# Autodesk Inventor assembly: Сборка1
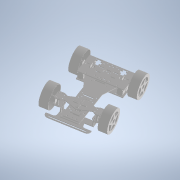
[picture p0: Inventor's stored thumbnail of the model, 180x180]
Saved by Autodesk Inventor 2022 (Build 260153000, 153)
## iProperties
Created: 2022-07-10
Part Number: Сборка1
Document SubType Name: Assembly
Designer: Константин
Author: Константин
## Documents named in this file (16)
- C:\Users\Константин\Desktop\практика галактика\Сборка1.iam
- C:\Users\Константин\Downloads\мотор.ipt
- C:\Users\Константин\Downloads\Рама.ipt
- C:\Users\Константин\Downloads\Ось.ipt
- C:\Users\Константин\Downloads\Крепеж.ipt
- C:\Users\Константин\Downloads\Звезда.ipt
- C:\Users\Константин\Downloads\Задняя часть.ipt
- C:\Users\Константин\Downloads\Бампер.ipt
- C:\Users\Константин\Downloads\m3x29.ipt
- C:\Users\Константин\Desktop\практика галактика\Колесо красивое.ipt
- C:\Users\Константин\Desktop\практика галактика\Крепеж колеса.ipt
- C:\Users\Константин\Desktop\практика галактика\Крепежная деталь.ipt
- C:\Users\Константин\Desktop\практика галактика\Кусок металла.ipt
- C:\Users\Константин\Desktop\практика галактика\Пластинка шасси.ipt
- C:\Users\Константин\Desktop\практика галактика\Сервопривод.ipt
- C:\Users\Константин\Desktop\практика галактика\Колесо красивое(для мотора).ipt
## Components (32 placed, 15 different names)
1. мотор:1 — Совмещение:61, Совмещение:62, Совмещение:63, Совмещение:64, Совмещение:65, Совмещение:72, Совмещение:79, Совмещение:80, Совмещение:81
2. Рама:1 — Совмещение:28, Совмещение:29, Совмещение:30, Угол:1, С поворотом:4, С поворотом:5, Совмещение:73, Совмещение:74, Совмещение:75
3. Ось:1 — Совмещение:1, Совмещение:27, Угол:1, Совмещение:50, С поворотом:1, Совмещение:51, Совмещение:55, Совмещение:56, Совмещение:57, Совмещение:58, Совмещение:59
4. Крепеж:1 — Совмещение:67, Совмещение:69, Совмещение:76, Совмещение:77
5. Звезда:1 — Совмещение:1, Совмещение:27, Совмещение:31, Совмещение:32
6. Задняя часть:1 — Совмещение:65, Совмещение:70, С поворотом:3, Совмещение:73, Совмещение:74, Совмещение:75, Угол:2
7. Бампер:1 — С поворотом:4, С поворотом:5
8. Крепеж колеса:1 — Совмещение:57, Совмещение:58, Совмещение:60, Совмещение:85
9. Сервопривод:1 — Совмещение:28, Совмещение:29, Совмещение:30, Совмещение:31, Совмещение:32
10. Крепежная деталь:2 — Совмещение:8, Совмещение:9, Совмещение:10, Совмещение:11, Совмещение:60
11. Кусок металла:4 — Совмещение:36, Совмещение:41, Совмещение:44, Совмещение:47
12. Кусок металла:5 — Совмещение:37, Совмещение:38, Совмещение:45, Совмещение:46
13. Кусок металла:7 — Совмещение:8, Совмещение:10
14. Кусок металла:9 — Совмещение:9, Совмещение:11
15. Крепежная деталь:3
16. Кусок металла:10 — Совмещение:35, Совмещение:39, Совмещение:43, Совмещение:49
17. Кусок металла:11 — Совмещение:34, Совмещение:40, Совмещение:42, Совмещение:48
18. Кусок металла:12 — Совмещение:50, С поворотом:1
19. Кусок металла:13 — Совмещение:51
20. Пластинка шасси:3 — Совмещение:34, Совмещение:35, Совмещение:36, Совмещение:37, Совмещение:38, Совмещение:39, Совмещение:40, Совмещение:41, Совмещение:42, Совмещение:43, Совмещение:44, Совмещение:45, Совмещение:46, Совмещение:47, Совмещение:48, Совмещение:49
21. Крепеж колеса:2 — Совмещение:55, Совмещение:56, Совмещение:59, Совмещение:87
22. Крепеж:2 — Совмещение:61, Совмещение:63
23. мотор:2 — Совмещение:66, Совмещение:67, Совмещение:68, Совмещение:69, Совмещение:70, Совмещение:82, Совмещение:83, Совмещение:84
24. Крепеж:3 — Совмещение:62, Совмещение:64, Совмещение:78
25. Крепеж:4 — Совмещение:66, Совмещение:68
26. m3x29:4 — Совмещение:72, Совмещение:78
27. Задняя часть:2 — С поворотом:3, Угол:2
28. m3x29:5 — Совмещение:76, Совмещение:77
29. Колесо красивое(для мотора):1 — Совмещение:79, Совмещение:80, Совмещение:81
30. Колесо красивое:1 — Совмещение:85
31. Колесо красивое(для мотора):2 — Совмещение:82, Совмещение:83, Совмещение:84, Заподлицо:1
32. Колесо красивое:2 — Совмещение:87, Заподлицо:1
## Relationships (79: Mate 68, CylindricalJoint 4, RevoluteJoint 4, Angle 2, Flush 1)
- Совмещение:1 [Mate]: Ось:1 ↔ Звезда:1
- [CylindricalJoint]: Крепежная деталь:2 ↔ Кусок металла:4
- [CylindricalJoint]: Крепежная деталь:2 ↔ Кусок металла:5
- [Mate]: Крепежная деталь:2 ↔ Кусок металла:5
- [Mate]: Крепежная деталь:2 ↔ Кусок металла:4
- Совмещение:8 [Mate]: Крепежная деталь:2 ↔ Кусок металла:7
- Совмещение:9 [Mate]: Крепежная деталь:2 ↔ Кусок металла:9
- Совмещение:10 [Mate]: Крепежная деталь:2 ↔ Кусок металла:7
- Совмещение:11 [Mate]: Крепежная деталь:2 ↔ Кусок металла:9
- [CylindricalJoint]: Крепежная деталь:3 ↔ Кусок металла:10
- [CylindricalJoint]: Крепежная деталь:3 ↔ Кусок металла:11
- [Mate]: Крепежная деталь:3 ↔ Кусок металла:11
- [Mate]: Крепежная деталь:3 ↔ Кусок металла:10
- [Mate]: Крепежная деталь:3 ↔ Кусок металла:12
- [Mate]: Крепежная деталь:3 ↔ Кусок металла:13
- [Mate]: Крепежная деталь:3 ↔ Кусок металла:12
- [Mate]: Крепежная деталь:3 ↔ Кусок металла:13
- Совмещение:27 [Mate]: Ось:1 ↔ Звезда:1
- Совмещение:28 [Mate]: Рама:1 ↔ Сервопривод:1
- Совмещение:29 [Mate]: Рама:1 ↔ Сервопривод:1
- Совмещение:30 [Mate]: Рама:1 ↔ Сервопривод:1
- Совмещение:31 [Mate]: Звезда:1 ↔ Сервопривод:1
- Совмещение:32 [Mate]: Звезда:1 ↔ Сервопривод:1
- Угол:1 [Angle] (0 deg): Рама:1 ↔ Ось:1
- Совмещение:34 [Mate]: Кусок металла:11 ↔ Пластинка шасси:3
- Совмещение:35 [Mate]: Кусок металла:10 ↔ Пластинка шасси:3
- Совмещение:36 [Mate]: Кусок металла:4 ↔ Пластинка шасси:3
- Совмещение:37 [Mate]: Кусок металла:5 ↔ Пластинка шасси:3
- Совмещение:38 [Mate]: Кусок металла:5 ↔ Пластинка шасси:3
- Совмещение:39 [Mate]: Кусок металла:10 ↔ Пластинка шасси:3
- Совмещение:40 [Mate]: Кусок металла:11 ↔ Пластинка шасси:3
- Совмещение:41 [Mate]: Кусок металла:4 ↔ Пластинка шасси:3
- Совмещение:42 [Mate]: Кусок металла:11 ↔ Пластинка шасси:3
- Совмещение:43 [Mate]: Кусок металла:10 ↔ Пластинка шасси:3
- Совмещение:44 [Mate]: Кусок металла:4 ↔ Пластинка шасси:3
- Совмещение:45 [Mate]: Кусок металла:5 ↔ Пластинка шасси:3
- Совмещение:46 [Mate]: Кусок металла:5 ↔ Пластинка шасси:3
- Совмещение:47 [Mate]: Кусок металла:4 ↔ Пластинка шасси:3
- Совмещение:48 [Mate]: Кусок металла:11 ↔ Пластинка шасси:3
- Совмещение:49 [Mate]: Кусок металла:10 ↔ Пластинка шасси:3
- Совмещение:50 [Mate]: Ось:1 ↔ Кусок металла:12
- С поворотом:1 [RevoluteJoint]: Ось:1 ↔ Кусок металла:12
- Совмещение:51 [Mate]: Ось:1 ↔ Кусок металла:13
- Совмещение:55 [Mate]: Ось:1 ↔ Крепеж колеса:2
- Совмещение:56 [Mate]: Ось:1 ↔ Крепеж колеса:2
- Совмещение:57 [Mate]: Ось:1 ↔ Крепеж колеса:1
- Совмещение:58 [Mate]: Ось:1 ↔ Крепеж колеса:1
- Совмещение:59 [Mate]: Ось:1 ↔ Крепеж колеса:2
- Совмещение:60 [Mate]: Крепеж колеса:1 ↔ Крепежная деталь:2
- Совмещение:61 [Mate]: мотор:1 ↔ Крепеж:2
- Совмещение:62 [Mate]: мотор:1 ↔ Крепеж:3
- Совмещение:63 [Mate]: мотор:1 ↔ Крепеж:2
- Совмещение:64 [Mate]: мотор:1 ↔ Крепеж:3
- Совмещение:65 [Mate]: мотор:1 ↔ Задняя часть:1
- Совмещение:66 [Mate]: мотор:2 ↔ Крепеж:4
- Совмещение:67 [Mate]: Крепеж:1 ↔ мотор:2
- Совмещение:68 [Mate]: мотор:2 ↔ Крепеж:4
- Совмещение:69 [Mate]: Крепеж:1 ↔ мотор:2
- Совмещение:70 [Mate]: Задняя часть:1 ↔ мотор:2
- Совмещение:72 [Mate]: мотор:1 ↔ m3x29:4
- С поворотом:3 [RevoluteJoint] (22 mm): Задняя часть:1 ↔ Задняя часть:2
- С поворотом:4 [RevoluteJoint]: Рама:1 ↔ Бампер:1
- С поворотом:5 [RevoluteJoint]: Рама:1 ↔ Бампер:1
- Совмещение:73 [Mate]: Рама:1 ↔ Задняя часть:1
- Совмещение:74 [Mate]: Рама:1 ↔ Задняя часть:1
- Совмещение:75 [Mate]: Рама:1 ↔ Задняя часть:1
- Угол:2 [Angle] (0 deg): Задняя часть:1 ↔ Задняя часть:2
- Совмещение:76 [Mate]: Крепеж:1 ↔ m3x29:5
- Совмещение:77 [Mate]: Крепеж:1 ↔ m3x29:5
- Совмещение:78 [Mate]: Крепеж:3 ↔ m3x29:4
- Совмещение:79 [Mate]: мотор:1 ↔ Колесо красивое(для мотора):1
- Совмещение:80 [Mate]: мотор:1 ↔ Колесо красивое(для мотора):1
- Совмещение:81 [Mate]: мотор:1 ↔ Колесо красивое(для мотора):1
- Совмещение:82 [Mate]: мотор:2 ↔ Колесо красивое(для мотора):2
- Совмещение:83 [Mate]: мотор:2 ↔ Колесо красивое(для мотора):2
- Совмещение:84 [Mate]: мотор:2 ↔ Колесо красивое(для мотора):2
- Совмещение:85 [Mate]: Крепеж колеса:1 ↔ Колесо красивое:1
- Совмещение:87 [Mate]: Крепеж колеса:2 ↔ Колесо красивое:2
- Заподлицо:1 [Flush]: Колесо красивое(для мотора):2 ↔ Колесо красивое:2
## Named parameters: d21_d19 = 0 mm, d22_d20 = 0 mm, d23_d4 = -51.921901 deg, d24_d5 = 0 mm, d25_d7 = 148.488223 deg, d26_d8 = 0 mm, d32_d21_d19 = 0 mm, d33_d22_d20 = 0 mm, d34_d23_d4 = -75.112645 deg, d35_d24_d5 = 0 mm, d36_d25_d7 = 124.867216 deg, d37_d26_d8 = 0 mm, d39_d28 = 0 mm, d40_d29 = 0 mm, d41_d30 = 0 mm, d42_d31 = 0 mm
